# Autodesk Inventor assembly: Assemblage_général
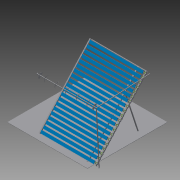
[picture p0: Inventor's stored thumbnail of the model, 180x180]
Saved by Autodesk Inventor 2015 SP1 (Build 190203100, 203)
## iProperties
Created: 2015-04-17
Part Number: Assemblage_général
Document SubType Name: Assembly
Designer: Cyril
Author: Cyril
## Documents named in this file (6)
- C:\Users\Cyril\Documents\OSE FR\Concentrateur solaire\Assemblage_général.iam
- C:\Users\Cyril\Documents\OSE FR\Concentrateur solaire\Assemblage_cadre-miroir.iam
- C:\Users\Cyril\Documents\OSE FR\Concentrateur solaire\Poutre.ipt
- C:\Users\Cyril\Documents\OSE FR\Concentrateur solaire\Sol.ipt
- C:\Users\Cyril\Documents\OSE FR\Concentrateur solaire\Pied.ipt
- C:\Users\Cyril\Documents\OSE FR\Concentrateur solaire\Absorbeur\Assemblage absorbeur.iam
## Components (6 placed, 5 different names)
1. Sol:1 — Mate:10, Mate:11, Flush:8, Mate:13, Mate:14
2. Poutre:2 — Mate:2, Flush:13, Mate:5, Mate:6, Flush:6, Angle:1, Mate:13, Mate:14
3. Pied:1 — Mate:5, Mate:6, Angle:1
4. Assemblage_cadre-miroir:1 [sub-assembly] — Mate:1, Flush:1, Flush:2
5. Assemblage_cadre-miroir:2 [sub-assembly] — Mate:1, Flush:1, Flush:2, Mate:2, Flush:13, Flush:6, Flush:7, Mate:9
6. Assemblage absorbeur:1 [sub-assembly] — Flush:7, Mate:9
## Relationships (16: Mate 9, Flush 6, Angle 1)
- Mate:1: Assemblage_cadre-miroir:1 ↔ Assemblage_cadre-miroir:2
- Flush:1: Assemblage_cadre-miroir:1 ↔ Assemblage_cadre-miroir:2
- Flush:2: Assemblage_cadre-miroir:1 ↔ Assemblage_cadre-miroir:2
- Mate:2: Poutre:2 ↔ Assemblage_cadre-miroir:2
- Flush:13: Poutre:2 ↔ Assemblage_cadre-miroir:2
- Mate:5: Poutre:2 ↔ Pied:1
- Mate:6: Poutre:2 ↔ Pied:1
- Flush:6 (350 mm): Poutre:2 ↔ Assemblage_cadre-miroir:2
- Angle:1 (240 deg): Poutre:2 ↔ Pied:1
- Flush:7: Assemblage_cadre-miroir:2 ↔ Assemblage absorbeur:1
- Mate:9 (1210 mm): Assemblage_cadre-miroir:2 ↔ Assemblage absorbeur:1
- Mate:10: Sol:1
- Mate:11: Sol:1
- Flush:8: Sol:1
- Mate:13: Sol:1 ↔ Poutre:2
- Mate:14 (-200 mm): Sol:1 ↔ Poutre:2
